# Autodesk Inventor assembly: Craftsman Socket U-Joint_2
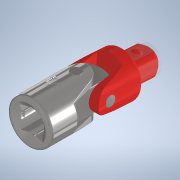
[picture p0: Inventor's stored thumbnail of the model, 180x180]
Saved by Autodesk Inventor 2021 (Build 250183000, 183)
## iProperties
Created: 2013-08-30
Part Number: Craftsman Socket U-Joint_2
Document SubType Name: Assembly
Designer: ASUS
Author: ASUS
## Documents named in this file (4)
- D:\Projects\P_Borewell\V2\Design\sps manipulator\Craftsman Socket U-Joint_2.iam
- D:\Projects\P_Borewell\V2\Design\sps manipulator\Craftsman Socket U-Joint Base.ipt
- D:\Projects\P_Borewell\V2\Design\sps manipulator\Craftsman Socket U-Joint Intermediate Body.ipt
- D:\Projects\P_Borewell\V2\Design\sps manipulator\Craftsman Socket U-Joint Drive.ipt
## Components (3 placed, 3 different names)
1. Craftsman Socket U-Joint Base:1 — Mate:1, Mate:2
2. Craftsman Socket U-Joint Intermediate Body:1 — Mate:1, Mate:2, Mate:3, Mate:4
3. Craftsman Socket U-Joint Drive:1 — Mate:3, Mate:4
## Relationships (4: Mate 4)
- Mate:1: Craftsman Socket U-Joint Base:1 ↔ Craftsman Socket U-Joint Intermediate Body:1
- Mate:2: Craftsman Socket U-Joint Base:1 ↔ Craftsman Socket U-Joint Intermediate Body:1
- Mate:3: Craftsman Socket U-Joint Intermediate Body:1 ↔ Craftsman Socket U-Joint Drive:1
- Mate:4: Craftsman Socket U-Joint Intermediate Body:1 ↔ Craftsman Socket U-Joint Drive:1
